# Autodesk Inventor assembly: Assembly1
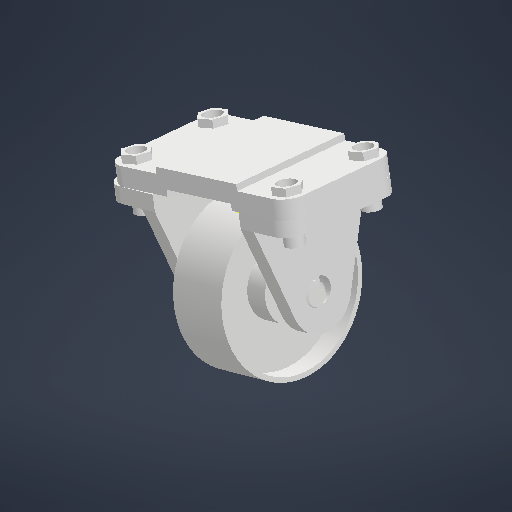
[picture p0: Inventor's stored thumbnail of the model, 512x512]
Saved by Autodesk Inventor 2026 (Build 300175000, 175)
## iProperties
Created: 2025-05-07
Part Number: Assembly1
Document SubType Name: Assembly
Designer: Ritul Kumari
Author: Ritul Kumari
## Documents named in this file (6)
- C:\Users\Ritul Kumari\Documents\Inventor\inventor P1\Assembly1.iam
- C:\Users\Ritul Kumari\Documents\Inventor\inventor P1\Part4.ipt
- C:\Users\Ritul Kumari\Documents\Inventor\inventor P1\Wheel.ipt
- C:\Users\Ritul Kumari\Documents\Inventor\inventor P1\axle support.ipt
- C:\Users\Ritul Kumari\Documents\Inventor\inventor P1\axle.ipt
- C:\Users\Ritul Kumari\Documents\Inventor\inventor P1\nut.ipt
## Components (9 placed, 5 different names)
1. Part4:1 — Insert:1, Insert:2, Insert:5, Insert:7, Insert:8, Insert:9
2. Wheel:1 — Insert:10
3. axle support:1 — Insert:2
4. axle support:2 — Insert:1
5. axle:1 — Insert:10
6. nut:2 — Insert:5
7. nut:4 — Insert:7
8. nut:5 — Insert:8
9. nut:6 — Insert:9
## Relationships (7: Insert 7)
- Insert:1: Part4:1 ↔ axle support:2
- Insert:2: Part4:1 ↔ axle support:1
- Insert:5: Part4:1 ↔ nut:2
- Insert:7: Part4:1 ↔ nut:4
- Insert:8: Part4:1 ↔ nut:5
- Insert:9: Part4:1 ↔ nut:6
- Insert:10: Wheel:1 ↔ axle:1
